# Autodesk Inventor assembly: HammerStick1
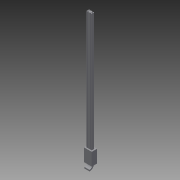
[picture p0: Inventor's stored thumbnail of the model, 180x180]
Saved by Autodesk Inventor 2015 (Build 190159000, 159)
## iProperties
Created: 2015-01-13
Part Number: HammerStick1
Document SubType Name: Assembly
Designer: harrykuperstein
Author: harrykuperstein
## Documents named in this file (3)
- C:\team3556-cad-2015\HammerStick1.iam
- C:\team3556-cad-2015\HammerStick Hook1.iam
- C:\team3556-cad-2015\HammerStick Stick.ipt
## Components (2 placed, 2 different names)
1. HammerStick Hook1:1 [sub-assembly] — Mate:1, Mate:2, Mate:3
2. HammerStick Stick:1 — Mate:1, Mate:2, Mate:3
## Relationships (3: Mate 3)
- Mate:1: HammerStick Hook1:1 ↔ HammerStick Stick:1
- Mate:2: HammerStick Hook1:1 ↔ HammerStick Stick:1
- Mate:3: HammerStick Hook1:1 ↔ HammerStick Stick:1
